# Autodesk Inventor assembly: 0505
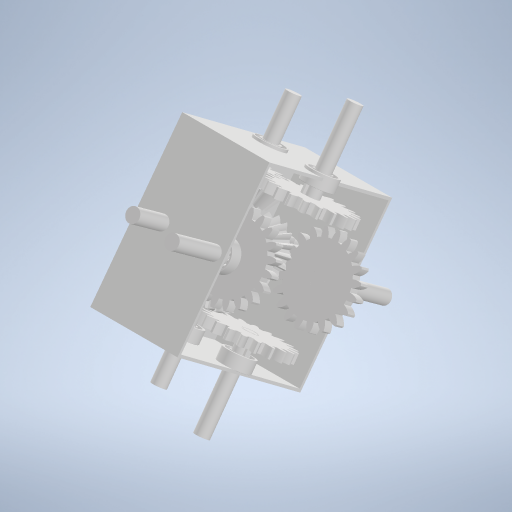
[picture p0: Inventor's stored thumbnail of the model, 512x512]
Saved by Autodesk Inventor 2023 (Build 270158000, 158)
## iProperties
Created: 2023-05-08
Part Number: 0505
Description: STEP AP203
Document SubType Name: Assembly
Designer: 310611102
Sending System: SolidWorks 2019
Preprocessor: SwSTEP 2.0
Title: 0505.STEP
Revision Number: ANY
## Documents named in this file (8)
- C:\Users\310611102\Documents\Inventor\SSR\avionics_2023ver\actuator_system\gearbox_ver1\0505.iam
- C:\Users\310611102\Documents\Inventor\SSR\avionics_2023ver\actuator_system\gearbox_ver1\ISO - Straight bevel gear 3M 36GT 18PT 20PA 20FW ---36O75H50MD16.0S_ISO - Straight bevel gear 3M 36GT 18PT 20PA 20FW ---36.ipt
- C:\Users\310611102\Documents\Inventor\SSR\avionics_2023ver\actuator_system\gearbox_ver1\straight bevel pinion_iso_ISO - Straight bevel pinion 3M18PT 36GT 20PA 20FW ---18O30H50MD15.0S1.ipt
- C:\Users\310611102\Documents\Inventor\SSR\avionics_2023ver\actuator_system\gearbox_ver1\ISO - Spur gear 4M 10T 20PA 10FW ---S10A75H50L15.0S1-1_ISO - Spur gear 4M 10T 20PA 10FW ---S10A75H50L15.0S1.ipt
- C:\Users\310611102\Documents\Inventor\SSR\avionics_2023ver\actuator_system\gearbox_ver1\ISO - Spur gear 4M 20T 20PA 10FW ---S20A75H50L15.0S1-1_ISO - Spur gear 4M 20T 20PA 10FW ---S20A75H50L15.0S1.ipt
- C:\Users\310611102\Documents\Inventor\SSR\avionics_2023ver\actuator_system\gearbox_ver1\±ì¤l.ipt
- C:\Users\310611102\Documents\Inventor\SSR\avionics_2023ver\actuator_system\gearbox_ver1\ISO 15 ABB - 3015 - 12,DE,NC,12_68-1_ISO 15 ABB - 3015 - 12,DE,NC,12_68.ipt
- C:\Users\310611102\Documents\Inventor\SSR\avionics_2023ver\actuator_system\gearbox_ver1\gearbox_box.ipt
## Components (30 placed, 30 different names)
1. ISO - Straight bevel gear 3M 36GT 18PT 20PA 20FW ---36O75H50MD16.0S_ISO - Straight bevel gear 3M 36GT 18PT 20PA 20FW ---36O75H50MD16.0S1_1
2. straight bevel pinion_iso_ISO - Straight bevel pinion 3M18PT 36GT 20PA 20FW ---18O30H50MD15.0S1_2
3. straight bevel pinion_iso_ISO - Straight bevel pinion 3M18PT 36GT 20PA 20FW ---18O30H50MD15.0S1_3
4. straight bevel pinion_iso_ISO - Straight bevel pinion 3M18PT 36GT 20PA 20FW ---18O30H50MD15.0S1_4
5. straight bevel pinion_iso_ISO - Straight bevel pinion 3M18PT 36GT 20PA 20FW ---18O30H50MD15.0S1_5
6. ISO - Spur gear 4M 10T 20PA 10FW ---S10A75H50L15.0S1-1_ISO - Spur gear 4M 10T 20PA 10FW ---S10A75H50L15.0S1_7
7. ISO - Spur gear 4M 20T 20PA 10FW ---S20A75H50L15.0S1-1_ISO - Spur gear 4M 20T 20PA 10FW ---S20A75H50L15.0S1_8
8. ISO - Spur gear 4M 10T 20PA 10FW ---S10A75H50L15.0S1-1_ISO - Spur gear 4M 10T 20PA 10FW ---S10A75H50L15.0S1_9
9. ISO - Spur gear 4M 10T 20PA 10FW ---S10A75H50L15.0S1-1_ISO - Spur gear 4M 10T 20PA 10FW ---S10A75H50L15.0S1_10
10. ISO - Spur gear 4M 10T 20PA 10FW ---S10A75H50L15.0S1-1_ISO - Spur gear 4M 10T 20PA 10FW ---S10A75H50L15.0S1_11
11. ISO - Spur gear 4M 20T 20PA 10FW ---S20A75H50L15.0S1-1_ISO - Spur gear 4M 20T 20PA 10FW ---S20A75H50L15.0S1_12
12. ISO - Spur gear 4M 20T 20PA 10FW ---S20A75H50L15.0S1-1_ISO - Spur gear 4M 20T 20PA 10FW ---S20A75H50L15.0S1_13
13. ISO - Spur gear 4M 20T 20PA 10FW ---S20A75H50L15.0S1-1_ISO - Spur gear 4M 20T 20PA 10FW ---S20A75H50L15.0S1_14
14. ±ì¤l_15
15. ±ì¤l_16
16. ±ì¤l_17
17. ±ì¤l_18
18. ±ì¤l_19
19. ±ì¤l_20
20. ±ì¤l_21
21. ±ì¤l_22
22. ISO 15 ABB - 3015 - 12,DE,NC,12_68-1_ISO 15 ABB - 3015 - 12,DE,NC,12_68_25
23. ISO 15 ABB - 3015 - 12,DE,NC,12_68-1_ISO 15 ABB - 3015 - 12,DE,NC,12_68_26
24. ISO 15 ABB - 3015 - 12,DE,NC,12_68-1_ISO 15 ABB - 3015 - 12,DE,NC,12_68_27
25. ISO 15 ABB - 3015 - 12,DE,NC,12_68-1_ISO 15 ABB - 3015 - 12,DE,NC,12_68_28
26. ISO 15 ABB - 3015 - 12,DE,NC,12_68-1_ISO 15 ABB - 3015 - 12,DE,NC,12_68_29
27. ISO 15 ABB - 3015 - 12,DE,NC,12_68-1_ISO 15 ABB - 3015 - 12,DE,NC,12_68_30
28. ISO 15 ABB - 3015 - 12,DE,NC,12_68-1_ISO 15 ABB - 3015 - 12,DE,NC,12_68_31
29. ISO 15 ABB - 3015 - 12,DE,NC,12_68-1_ISO 15 ABB - 3015 - 12,DE,NC,12_68_32
30. gearbox_box:1 — Mate:1
## Relationships (1: Mate 1)
- Mate:1: gearbox_box:1
